# Autodesk Inventor assembly: Assembly1
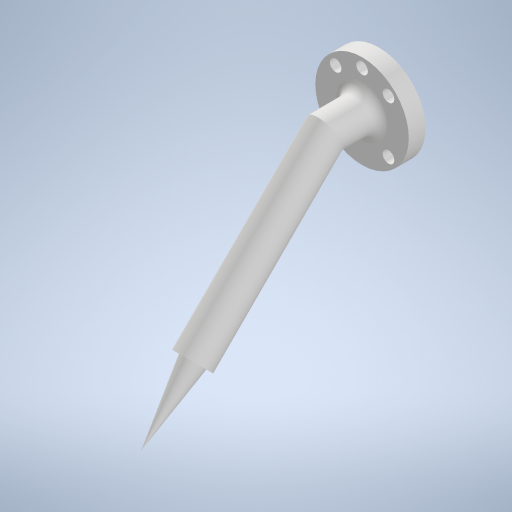
[picture p0: Inventor's stored thumbnail of the model, 512x512]
Saved by Autodesk Inventor 2024.2 (Build 282272000, 272)
## iProperties
Created: 2024-03-13
Part Number: Assembly1
Document SubType Name: Assembly
Designer: parmo
Author: parmo
## Documents named in this file (3)
- C:\Users\parmo\OneDrive\Escritorio\TrabajosUN\Robótica\Laboratorios\Laboratorio 1\Assembly1.iam
- C:\Users\parmo\OneDrive\Escritorio\TrabajosUN\Robótica\Laboratorios\Laboratorio 1\PenTool.ipt
- C:\Users\parmo\OneDrive\Escritorio\TrabajosUN\Robótica\Laboratorios\Laboratorio 1\Tip.ipt
## Components (2 placed, 2 different names)
1. PenTool:1 — Rotational:1
2. Tip:1 — Rotational:1
## Relationships (1: RevoluteJoint 1)
- Rotational:1 [RevoluteJoint]: PenTool:1 ↔ Tip:1
